# Autodesk Inventor assembly: A2017_T4_12
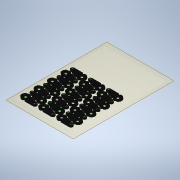
[picture p0: Inventor's stored thumbnail of the model, 180x180]
Saved by Autodesk Inventor 2020 (Build 240168000, 168)
## iProperties
Created: 2021-08-27
Part Number: A2017_T4_12
Document SubType Name: Assembly
Designer: Masato
Author: Masato
## Documents named in this file (3)
- C:\Inventor\SUSTAINA-OP\Cam\A2017_T4_12.iam
- C:\Inventor\SUSTAINA-OP\Cam\DisposableBoard.ipt
- C:\Inventor\SUSTAINA-OP\LowerBody\Ankle\Ankle_side_pitch_frame.ipt
## Components (25 placed, 2 different names)
1. DisposableBoard:1 — メイト:2, メイト:1, フラッシュ:1, フラッシュ:2, メイト:4, フラッシュ:3, 正接:1, メイト:5, 正接:2
2. Ankle_side_pitch_frame:1 — メイト:4, フラッシュ:3, 正接:1, メイト:6
3. Ankle_side_pitch_frame:2 — メイト:5, メイト:6, 正接:2
4. Ankle_side_pitch_frame:3
5. Ankle_side_pitch_frame:4
6. Ankle_side_pitch_frame:5
7. Ankle_side_pitch_frame:6
8. Ankle_side_pitch_frame:7
9. Ankle_side_pitch_frame:8
10. Ankle_side_pitch_frame:9
11. Ankle_side_pitch_frame:10
12. Ankle_side_pitch_frame:11
13. Ankle_side_pitch_frame:12
14. Ankle_side_pitch_frame:13
15. Ankle_side_pitch_frame:14
16. Ankle_side_pitch_frame:15
17. Ankle_side_pitch_frame:16
18. Ankle_side_pitch_frame:17
19. Ankle_side_pitch_frame:18
20. Ankle_side_pitch_frame:19
21. Ankle_side_pitch_frame:20
22. Ankle_side_pitch_frame:21
23. Ankle_side_pitch_frame:22
24. Ankle_side_pitch_frame:23
25. Ankle_side_pitch_frame:24
## Component patterns: (12 elements, first: Ankle_side_pitch_frame:1 + Ankle_side_pitch_frame:2)
## Relationships (10: Mate 5, Flush 3, Tangent 2)
- メイト:2 [Mate]: DisposableBoard:1
- メイト:1 [Mate]: DisposableBoard:1
- フラッシュ:1 [Flush]: DisposableBoard:1
- フラッシュ:2 [Flush]: DisposableBoard:1
- メイト:4 [Mate]: DisposableBoard:1 ↔ Ankle_side_pitch_frame:1
- フラッシュ:3 [Flush] (12 mm): DisposableBoard:1 ↔ Ankle_side_pitch_frame:1
- 正接:1 [Tangent] (2 mm): DisposableBoard:1 ↔ Ankle_side_pitch_frame:1
- メイト:5 [Mate]: DisposableBoard:1 ↔ Ankle_side_pitch_frame:2
- メイト:6 [Mate] (2.5 mm): Ankle_side_pitch_frame:1 ↔ Ankle_side_pitch_frame:2
- 正接:2 [Tangent] (8 mm): DisposableBoard:1 ↔ Ankle_side_pitch_frame:2
